# Autodesk Inventor assembly: FULL SWERVE DRIVE ASSEMBLY!  6!
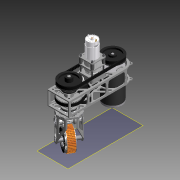
[picture p0: Inventor's stored thumbnail of the model, 180x180]
Saved by Autodesk Inventor 2012 (Build 160160000, 160)
## iProperties
Created: 2013-11-03
Part Number: FULL SWERVE DRIVE ASSEMBLY!  6!
Document SubType Name: Assembly
Designer: Bryce
Author: Bryce
## Documents named in this file (16)
- C:\Users\Bryce\Dropbox\Inventor Design Project Files\Independent Swerves\Inventor 2012\FULL SWERVE DRIVE ASSEMBLY!  6!.iam
- C:\Users\Bryce\Dropbox\Inventor Design Project Files\Independent Swerves\Inventor 2012\upper gearbox frame 5.ipt
- C:\Users\Bryce\Dropbox\Inventor Design Project Files\Independent Swerves\Inventor 2012\collar bearing systom.ipt
- C:\Users\Bryce\Dropbox\Inventor Design Project Files\Independent Swerves\Inventor 2012\Lower box main assembly 6.iam
- C:\Users\Bryce\Dropbox\Inventor Design Project Files\Independent Swerves\Imported Components\CIM Motor.iam
- C:\Users\Bryce\Dropbox\Inventor Design Project Files\Independent Swerves\Imported Components\BD Gearbox and Bracket Assy 4.iam
- C:\Users\Bryce\Dropbox\Inventor Design Project Files\Independent Swerves\Inventor 2012\turn encoder assembly 2.iam
- C:\Users\Bryce\Dropbox\Inventor Design Project Files\Independent Swerves\Inventor 2012\drive encoder assembly.iam
- C:\Users\Bryce\Dropbox\Inventor Design Project Files\Independent Swerves\Inventor 2012\2.25 U frame.ipt
- C:\Users\Bryce\Dropbox\Inventor Design Project Files\Independent Swerves\Imported Components\encoder gear turn small.ipt
- C:\Users\Bryce\Dropbox\Inventor Design Project Files\Independent Swerves\Imported Components\15T plastick sprocket .375 threaded.ipt
- C:\Users\Bryce\Dropbox\Inventor Design Project Files\Independent Swerves\Imported Components\encoder gear small 2.ipt
- C:\Users\Bryce\Dropbox\Inventor Design Project Files\Independent Swerves\Imported Components\drive spocket 40t.ipt
- C:\Users\Bryce\Dropbox\Inventor Design Project Files\Independent Swerves\Imported Components\large drive belt.ipt
- C:\Users\Bryce\Dropbox\Inventor Design Project Files\Independent Swerves\Inventor 2012\short turn belt.ipt
- C:\Users\Bryce\Dropbox\Inventor Design Project Files\Independent Swerves\Imported Components\turn spocket 44t Al.ipt
## Components (17 placed, 15 different names)
1. upper gearbox frame 5:1 — Mate:1, Insert:1, Insert:2, Mate:3, Mate:4, Mate:5, Mate:6, Mate:7, Mate:8, Mate:9, Mate:10, Insert:4, Insert:5, Mate:11, Mate:12, Flush:1, Angle:1, Angle:2, Angle:3
2. Lower box main assembly 6:1 [sub-assembly] — Mate:1, Mate:2, Mate:13, Flush:3, Insert:7, Flush:6, Mate:18, Flush:9, Tangent:1
3. collar bearing systom:1 — Insert:2, Mate:2
4. collar bearing systom:2 — Insert:1
5. CIM Motor:1 [sub-assembly] — Mate:3, Mate:4, Mate:5, Mate:6, Mate:7, Mate:15
6. BD Gearbox and Bracket Assy 4:1 [sub-assembly] — Mate:8, Mate:9, Mate:10, Insert:6
7. turn encoder assembly 2:2 [sub-assembly] — Insert:4, Flush:2, Rotation:1, Angle:1
8. drive encoder assembly:1 [sub-assembly] — Insert:5, Angle:2, Rotation:3
9. 2.25 U frame:1 — Mate:11, Mate:12, Flush:1
10. encoder gear turn small:1 — Mate:13, Flush:2, Flush:3, Rotation:1
11. turn spocket 44t Al:1 — Mate:18, Flush:8, Flush:9, Rotation:5
12. 15T plastick sprocket .375 threaded:1 — Insert:6, Insert:10, Flush:8, Rotation:5
13. encoder gear small 2:1 — Insert:7, Rotation:3, Flush:6, Insert:8
14. drive spocket 40t:1 — Insert:8, Flush:7, Mate:16, Rotation:4
15. drive spocket 40t:2 — Mate:15, Flush:7, Insert:9, Rotation:4
16. large drive belt:1 — Insert:9, Mate:16
17. short turn belt:1 — Insert:10
## Relationships (41: Mate 17, Insert 9, Flush 7, RelateRotation 4, Angle 3, Tangent 1)
- Mate:1: upper gearbox frame 5:1 ↔ Lower box main assembly 6:1
- Insert:1: upper gearbox frame 5:1 ↔ collar bearing systom:2
- Insert:2: upper gearbox frame 5:1 ↔ collar bearing systom:1
- Mate:2 (1.5875 mm): Lower box main assembly 6:1 ↔ collar bearing systom:1
- Mate:3: upper gearbox frame 5:1 ↔ CIM Motor:1
- Mate:4 (6.35 mm): upper gearbox frame 5:1 ↔ CIM Motor:1
- Mate:5 (6.35 mm): upper gearbox frame 5:1 ↔ CIM Motor:1
- Mate:6 (6.35 mm): upper gearbox frame 5:1 ↔ CIM Motor:1
- Mate:7 (6.35 mm): upper gearbox frame 5:1 ↔ CIM Motor:1
- Mate:8: upper gearbox frame 5:1 ↔ BD Gearbox and Bracket Assy 4:1
- Mate:9 (6.35 mm): upper gearbox frame 5:1 ↔ BD Gearbox and Bracket Assy 4:1
- Mate:10 (6.35 mm): upper gearbox frame 5:1 ↔ BD Gearbox and Bracket Assy 4:1
- Insert:4: upper gearbox frame 5:1 ↔ turn encoder assembly 2:2
- Insert:5: upper gearbox frame 5:1 ↔ drive encoder assembly:1
- Mate:11: upper gearbox frame 5:1 ↔ 2.25 U frame:1
- Mate:12: upper gearbox frame 5:1 ↔ 2.25 U frame:1
- Flush:1: upper gearbox frame 5:1 ↔ 2.25 U frame:1
- Mate:13: Lower box main assembly 6:1 ↔ encoder gear turn small:1
- Flush:2: turn encoder assembly 2:2 ↔ encoder gear turn small:1
- Flush:3: Lower box main assembly 6:1 ↔ encoder gear turn small:1
- Insert:6 (1.5875 mm): BD Gearbox and Bracket Assy 4:1 ↔ 15T plastick sprocket .375 threaded:1
- Rotation:1 [RelateRotation] (1 ul): turn encoder assembly 2:2 ↔ encoder gear turn small:1
- Angle:1 (0 deg): upper gearbox frame 5:1 ↔ turn encoder assembly 2:2
- Angle:2 (0 deg): upper gearbox frame 5:1 ↔ drive encoder assembly:1
- Insert:7: Lower box main assembly 6:1 ↔ encoder gear small 2:1
- Rotation:3 [RelateRotation] (1 ul): drive encoder assembly:1 ↔ encoder gear small 2:1
- Flush:6: Lower box main assembly 6:1 ↔ encoder gear small 2:1
- Insert:8 (1.5875 mm): encoder gear small 2:1 ↔ drive spocket 40t:1
- Mate:15: CIM Motor:1 ↔ drive spocket 40t:2
- Flush:7: drive spocket 40t:1 ↔ drive spocket 40t:2
- Insert:9 (1 mm): drive spocket 40t:2 ↔ large drive belt:1
- Mate:16 (31.2674 mm): drive spocket 40t:1 ↔ large drive belt:1
- Rotation:4 [RelateRotation] (1 ul): drive spocket 40t:1 ↔ drive spocket 40t:2
- Insert:10 (1 mm): 15T plastick sprocket .375 threaded:1 ↔ short turn belt:1
- [Mate] (34.4424 mm): turn spocket 44t Al:1 ↔ short turn belt:1
- Mate:18: Lower box main assembly 6:1 ↔ turn spocket 44t Al:1
- Flush:8: turn spocket 44t Al:1 ↔ 15T plastick sprocket .375 threaded:1
- Flush:9: Lower box main assembly 6:1 ↔ turn spocket 44t Al:1
- Rotation:5 [RelateRotation] (3 ul): turn spocket 44t Al:1 ↔ 15T plastick sprocket .375 threaded:1
- Angle:3 (0 deg): upper gearbox frame 5:1
- Tangent:1: Lower box main assembly 6:1
